# Autodesk Inventor assembly: gripper_assem
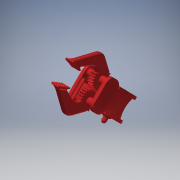
[picture p0: Inventor's stored thumbnail of the model, 180x180]
Saved by Autodesk Inventor 2018.2 (Build 222227000, 227)
## iProperties
Created: 2014-04-25
Part Number: gripper_assem
Document SubType Name: Assembly
Designer: t_emanb
Author: t_emanb
## Documents named in this file (7)
- C:\Users\mcnameed\git\carrickdojo\3D Printing\RoboticArm\gripper_assem.iam
- C:\Users\mcnameed\git\carrickdojo\3D Printing\RoboticArm\upper_pin.ipt
- C:\Users\mcnameed\git\carrickdojo\3D Printing\RoboticArm\upper_servo.ipt
- C:\Users\mcnameed\git\carrickdojo\3D Printing\RoboticArm\gripper_gearMirror.ipt
- C:\Users\mcnameed\git\carrickdojo\3D Printing\RoboticArm\gripper_base2.ipt
- C:\Users\mcnameed\git\carrickdojo\3D Printing\RoboticArm\gripper_base.ipt
- C:\Users\mcnameed\git\carrickdojo\3D Printing\RoboticArm\gripper_gearServo.ipt
## Components (6 placed, 5 different names)
1. upper_servo:1 — Flush:5, Mate:29, Mate:36
2. upper_pin:1 — Flush:1, Flush:2, Mate:17, Flush:3, Mate:26, Mate:35
3. Spur Gear1:2 — Mate:19, Mate:20
4. gripper_base2:1 — Flush:1, Flush:2, Mate:17, Mate:19, Mate:20
5. gripper_base:1 — Flush:3, Mate:26, Flush:5, Mate:29, Mate:35, Mate:36
6. Spur Gear1:3
## Relationships (11: Mate 7, Flush 4)
- Flush:1: upper_pin:1 ↔ gripper_base2:1
- Flush:2: upper_pin:1 ↔ gripper_base2:1
- Mate:17: upper_pin:1 ↔ gripper_base2:1
- Mate:19: Spur Gear1:2 ↔ gripper_base2:1
- Mate:20: Spur Gear1:2 ↔ gripper_base2:1
- Flush:3: upper_pin:1 ↔ gripper_base:1
- Mate:26: upper_pin:1 ↔ gripper_base:1
- Flush:5: upper_servo:1 ↔ gripper_base:1
- Mate:29: upper_servo:1 ↔ gripper_base:1
- Mate:35: upper_pin:1 ↔ gripper_base:1
- Mate:36: upper_servo:1 ↔ gripper_base:1
